# Autodesk Inventor assembly: Ensamblaje_completo
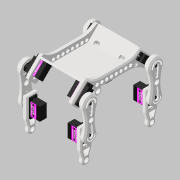
[picture p0: Inventor's stored thumbnail of the model, 180x180]
Saved by Autodesk Inventor 2022.2 (Build 262287010, 287A)
## iProperties
Created: 2022-06-14
Part Number: Ensamblaje_completo
Document SubType Name: Assembly
Designer: Usuario
Author: Usuario
## Documents named in this file (6)
- D:\Users\Usuario\Documents\Inventor\Aston\Ensamblaje_completo.iam
- D:\Users\Usuario\Documents\Inventor\Aston\Chassis_V2.ipt
- D:\Users\Usuario\Documents\Inventor\Aston\Soporte_electronica.ipt
- D:\Users\Usuario\Documents\Inventor\Aston\MG90S.ipt
- D:\Users\Usuario\Documents\Inventor\Aston\Femur_V2.ipt
- D:\Users\Usuario\Documents\Inventor\Aston\Tibia_V2.ipt
## Components (19 placed, 5 different names)
1. Chassis_V2:1 — Nivelación:1, Coincidencia:1, Nivelación:2, Coincidencia:3, Coincidencia:4, Coincidencia:5, Coincidencia:6
2. Soporte_electronica:1 — Nivelación:1, Coincidencia:1, Nivelación:2, Coincidencia:2
3. Chassis_V2:3 — Coincidencia:2, Coincidencia:7, Coincidencia:8, Coincidencia:9, Coincidencia:10
4. MG90S:2 — Coincidencia:3, Coincidencia:4, Coincidencia:11
5. MG90S:3 — Coincidencia:5, Coincidencia:6, Coincidencia:12
6. MG90S:4 — Coincidencia:9, Coincidencia:10, Coincidencia:14
7. MG90S:5 — Coincidencia:7, Coincidencia:8, Coincidencia:13
8. Femur_V2:2 — Coincidencia:13, Coincidencia:22
9. Femur_V2:3 — Coincidencia:14, Coincidencia:21
10. Femur_V2:4 — Coincidencia:11, Coincidencia:20
11. Femur_V2:5 — Coincidencia:12, Coincidencia:19
12. Tibia_V2:1 — Coincidencia:18
13. Tibia_V2:2 — Coincidencia:17
14. Tibia_V2:3 — Coincidencia:15
15. Tibia_V2:4 — Coincidencia:16
16. MG90S:6 — Coincidencia:18, Coincidencia:20
17. MG90S:7 — Coincidencia:17, Coincidencia:19
18. MG90S:8 — Coincidencia:16, Coincidencia:21
19. MG90S:9 — Coincidencia:15, Coincidencia:22
## Relationships (24: Mate 22, Flush 2)
- Nivelación:1 [Flush]: Chassis_V2:1 ↔ Soporte_electronica:1
- Coincidencia:1 [Mate]: Chassis_V2:1 ↔ Soporte_electronica:1
- Nivelación:2 [Flush]: Chassis_V2:1 ↔ Soporte_electronica:1
- Coincidencia:2 [Mate]: Soporte_electronica:1 ↔ Chassis_V2:3
- Coincidencia:3 [Mate]: Chassis_V2:1 ↔ MG90S:2
- Coincidencia:4 [Mate]: Chassis_V2:1 ↔ MG90S:2
- Coincidencia:5 [Mate]: Chassis_V2:1 ↔ MG90S:3
- Coincidencia:6 [Mate]: Chassis_V2:1 ↔ MG90S:3
- Coincidencia:7 [Mate]: Chassis_V2:3 ↔ MG90S:5
- Coincidencia:8 [Mate]: Chassis_V2:3 ↔ MG90S:5
- Coincidencia:9 [Mate]: Chassis_V2:3 ↔ MG90S:4
- Coincidencia:10 [Mate]: Chassis_V2:3 ↔ MG90S:4
- Coincidencia:11 [Mate]: MG90S:2 ↔ Femur_V2:4
- Coincidencia:12 [Mate]: MG90S:3 ↔ Femur_V2:5
- Coincidencia:13 [Mate]: MG90S:5 ↔ Femur_V2:2
- Coincidencia:14 [Mate]: MG90S:4 ↔ Femur_V2:3
- Coincidencia:15 [Mate]: Tibia_V2:3 ↔ MG90S:9
- Coincidencia:16 [Mate]: Tibia_V2:4 ↔ MG90S:8
- Coincidencia:17 [Mate]: Tibia_V2:2 ↔ MG90S:7
- Coincidencia:18 [Mate]: Tibia_V2:1 ↔ MG90S:6
- Coincidencia:19 [Mate]: Femur_V2:5 ↔ MG90S:7
- Coincidencia:20 [Mate]: Femur_V2:4 ↔ MG90S:6
- Coincidencia:21 [Mate]: Femur_V2:3 ↔ MG90S:8
- Coincidencia:22 [Mate]: Femur_V2:2 ↔ MG90S:9
